# Autodesk Inventor assembly: MiddleShaftAssembly
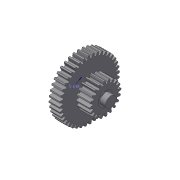
[picture p0: Inventor's stored thumbnail of the model, 180x180]
Saved by Autodesk Inventor 2013 SP1 (Build 170176100, 176)
## iProperties
Created: 2013-12-03
Part Number: MiddleShaftAssembly
Document SubType Name: Assembly
Designer: robotics
Author: robotics
## Documents named in this file (4)
- C:\Users\robotics\Documents\GitHub\2014-Preseason-Single-Speed-Gearbox\manufacture\assemblies\MiddleShaftAssembly.iam
- C:\Users\robotics\Documents\GitHub\2014-Preseason-Single-Speed-Gearbox\buy\VexPro\Gears\217-2701-STEP\Imported Components\217-2701.20121204\217-2701.20121204.ipt
- C:\Users\robotics\Documents\GitHub\2014-Preseason-Single-Speed-Gearbox\buy\VexPro\Gears\217-2707-STEP\Imported Components\217-2707.20121204\217-2707.20121204.ipt
- C:\Users\robotics\Documents\GitHub\2014-Preseason-Single-Speed-Gearbox\manufacture\parts\Shaft\MiddleShaft.ipt
## Components (3 placed, 3 different names)
1. 217-2701.20121204:1 — Flush:5
2. 217-2707.20121204:1 — Flush:6
3. MiddleShaft:1 — Flush:5, Flush:6
## Relationships (6: Mate 4, Flush 2)
- [Mate]: 217-2707.20121204:1 ↔ MiddleShaft:1
- [Mate]: 217-2707.20121204:1 ↔ MiddleShaft:1
- [Mate]: 217-2701.20121204:1 ↔ MiddleShaft:1
- [Mate]: 217-2701.20121204:1 ↔ MiddleShaft:1
- Flush:5: 217-2701.20121204:1 ↔ MiddleShaft:1
- Flush:6: 217-2707.20121204:1 ↔ MiddleShaft:1
